# Autodesk Inventor assembly: Ensamblaje2
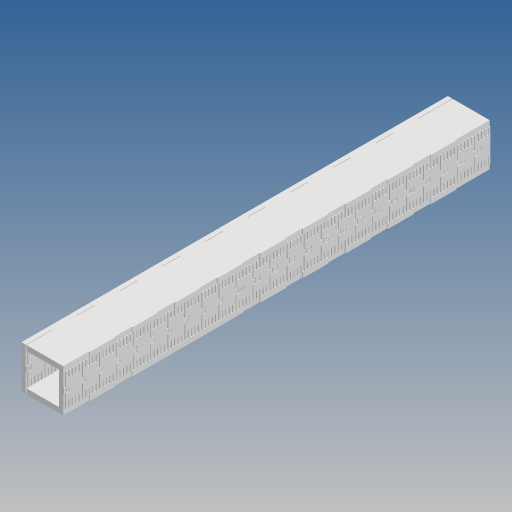
[picture p0: Inventor's stored thumbnail of the model, 512x512]
Saved by Autodesk Inventor 2024 (Build 280153000, 153)
## iProperties
Created: 2024-05-31
Part Number: Ensamblaje2
Document SubType Name: Assembly
Designer: Pablo
Author: Pablo
## Documents named in this file (3)
- D:\Users\Pablo\Desktop\UVG\otros\TesisM\Ensamblaje2.iam
- D:\Users\Pablo\Desktop\UVG\otros\TesisM\Pieza4.ipt
- D:\Users\Pablo\Desktop\UVG\otros\TesisM\Pieza5.ipt
## Components (4 placed, 2 different names)
1. Pieza4:1 — Nivelación:1, Nivelación:2, Nivelación:5, Nivelación:6, Coincidencia:3
2. Pieza4:2 — Nivelación:3, Nivelación:4, Coincidencia:1, Coincidencia:2
3. Pieza5:1 — Nivelación:1, Nivelación:2, Nivelación:3, Nivelación:4, Coincidencia:1, Coincidencia:3
4. Pieza5:2 — Nivelación:5, Nivelación:6, Coincidencia:2
## Relationships (9: Flush 6, Mate 3)
- Nivelación:1 [Flush]: Pieza4:1 ↔ Pieza5:1
- Nivelación:2 [Flush]: Pieza4:1 ↔ Pieza5:1
- Nivelación:3 [Flush]: Pieza4:2 ↔ Pieza5:1
- Nivelación:4 [Flush]: Pieza4:2 ↔ Pieza5:1
- Coincidencia:1 [Mate]: Pieza4:2 ↔ Pieza5:1
- Nivelación:5 [Flush]: Pieza4:1 ↔ Pieza5:2
- Nivelación:6 [Flush]: Pieza4:1 ↔ Pieza5:2
- Coincidencia:2 [Mate]: Pieza4:2 ↔ Pieza5:2
- Coincidencia:3 [Mate]: Pieza4:1 ↔ Pieza5:1
